# Autodesk Inventor assembly: corners bottom
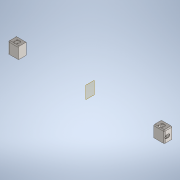
[picture p0: Inventor's stored thumbnail of the model, 180x180]
Saved by Autodesk Inventor 2020 (Build 240168000, 168)
## iProperties
Created: 2022-11-18
Part Number: corners bottom
Document SubType Name: Assembly
Designer: super
Author: super
## Documents named in this file (3)
- C:\desk\promissionsave\inventor\container\corners top.iam
- C:\desk\promissionsave\inventor\container\corner_TL.ipt
- C:\desk\promissionsave\inventor\container\corner_TL_MIR.ipt
## Components (2 placed, 2 different names)
1. corner_TL:1 — Flush:1
2. corner_TL_MIR:1 — Mate:1
## Relationships (2: Flush 1, Mate 1)
- Flush:1 (1057.2 mm): corner_TL:1
- Mate:1 (1057.2 mm): corner_TL_MIR:1
